# Autodesk Inventor assembly: Montagem_sistema
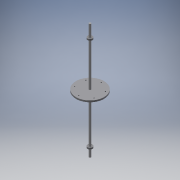
[picture p0: Inventor's stored thumbnail of the model, 180x180]
Saved by Autodesk Inventor 2018 (Build 220112000, 112)
## iProperties
Created: 2019-03-28
Part Number: Montagem_sistema
Material: Genérico
Document SubType Name: Assembly
Designer: vinig
Author: vinig
## Documents named in this file (4)
- C:\Users\vinig\OneDrive\Ambiente de Trabalho\Vinícius\TCC\Computacional\Montagem_sistema.iam
- C:\Users\vinig\OneDrive\Ambiente de Trabalho\Vinícius\TCC\Computacional\Disco.ipt
- C:\Users\vinig\OneDrive\Ambiente de Trabalho\Vinícius\TCC\Computacional\Eixo.ipt
- C:\Users\vinig\OneDrive\Ambiente de Trabalho\Vinícius\TCC\Computacional\Rolamento_6201_ZZ\6201-2Z.iam
## Components (4 placed, 3 different names)
1. Disco:1 — Rígida:1
2. Eixo:1 — Cilíndrica:1, Cilíndrica:2, Alinhamento:1, Rígida:1
3. 6201-2Z:1 [sub-assembly] — Cilíndrica:1, Alinhamento:1, Coincidência:1, Coincidência:2
4. 6201-2Z:2 [sub-assembly] — Cilíndrica:2, Coincidência:1, Coincidência:2
## Relationships (6: CylindricalJoint 2, Mate 2, Flush 1, WeldJoint 1)
- Cilíndrica:1 [CylindricalJoint]: Eixo:1 ↔ 6201-2Z:1
- Cilíndrica:2 [CylindricalJoint]: Eixo:1 ↔ 6201-2Z:2
- Alinhamento:1 [Flush] (52 mm): Eixo:1 ↔ 6201-2Z:1
- Coincidência:1 [Mate] (600 mm): 6201-2Z:1 ↔ 6201-2Z:2
- Coincidência:2 [Mate] (600 mm): 6201-2Z:1 ↔ 6201-2Z:2
- Rígida:1 [WeldJoint]: Disco:1 ↔ Eixo:1
